# Autodesk Inventor assembly: Gamepad_Left
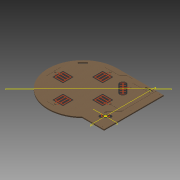
[picture p0: Inventor's stored thumbnail of the model, 180x180]
Saved by Autodesk Inventor 2014 SP1 (Build 180222100, 222)
## iProperties
Created: 2014-02-22
Part Number: Gamepad_Left
Document SubType Name: Assembly
Designer: tuleu
Author: tuleu
## Documents named in this file (6)
- C:\Users\tuleu\Documents\giant-snes-gamepad\cad\Gamepad_Left.iam
- C:\Users\tuleu\Documents\giant-snes-gamepad\cad\Base_Left.ipt
- C:\Users\tuleu\Documents\giant-snes-gamepad\cad\Square_Cell.iam
- C:\Users\tuleu\Documents\giant-snes-gamepad\cad\Trigger_Cell.iam
- C:\Users\tuleu\Documents\giant-snes-gamepad\cad\Start_Cell.iam
- C:\Users\tuleu\Documents\giant-snes-gamepad\cad\Foam_Left.ipt
## Components (8 placed, 5 different names)
1. Base_Left:1 — Flush:3, Flush:4
2. Square_Cell:1 [sub-assembly]
3. Square_Cell:2 [sub-assembly]
4. Square_Cell:3 [sub-assembly]
5. Square_Cell:4 [sub-assembly]
6. Trigger_Cell:1 [sub-assembly]
7. Start_Cell:1 [sub-assembly]
8. Foam_Left:1 — Flush:3, Flush:4
## Relationships (18: Mate 12, Flush 4, Symmetry 2)
- [Mate]: Base_Left:1 ↔ Square_Cell:2
- [Mate]: Base_Left:1 ↔ Square_Cell:3
- [Mate]: Base_Left:1 ↔ Square_Cell:1
- [Mate]: Base_Left:1 ↔ Square_Cell:4
- [Mate]: Square_Cell:1 ↔ Square_Cell:3
- [Flush]: Square_Cell:2 ↔ Square_Cell:4
- [Symmetry]: Square_Cell:2 ↔ Square_Cell:4
- [Symmetry]: Square_Cell:1 ↔ Square_Cell:3
- [Mate]: Base_Left:1 ↔ Square_Cell:1
- [Mate]: Base_Left:1 ↔ Square_Cell:4
- [Mate] (205 mm): Base_Left:1 ↔ Square_Cell:4
- [Mate]: Base_Left:1 ↔ Trigger_Cell:1
- [Flush]: Base_Left:1 ↔ Trigger_Cell:1
- [Mate] (-400 mm): Base_Left:1 ↔ Trigger_Cell:1
- [Mate]: Base_Left:1 ↔ Start_Cell:1
- [Mate]: Base_Left:1 ↔ Start_Cell:1
- Flush:3: Base_Left:1 ↔ Foam_Left:1
- Flush:4: Base_Left:1 ↔ Foam_Left:1
